# Autodesk Inventor assembly: WheelStrutLocomotion
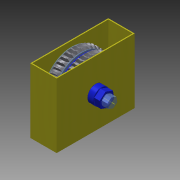
[picture p0: Inventor's stored thumbnail of the model, 180x180]
Saved by Autodesk Inventor 2014 (Build 180170000, 170)
## iProperties
Created: 2014-08-24
Part Number: WheelStrutLocomotion
Document SubType Name: Assembly
Designer: sam
Author: sam
## Documents named in this file (9)
- C:\Users\sam\Desktop\Octanis1-CAD\AI\WheelStrutLocomotion.iam
- C:\Users\sam\Desktop\Octanis1-CAD\AI\WheelStrutLocomotion\Design Accelerator\Shaft1.iam
- C:\Users\sam\Desktop\Octanis1-CAD\AI\WheelStrutLocomotion\Design Accelerator\Shaft3.iam
- C:\Users\sam\Desktop\Octanis1-CAD\AI\WheelStrutLocomotion\Design Accelerator\Worm Gears2.iam
- C:\Users\sam\Desktop\Octanis1-CAD\AI\WheelStrutLocomotion\Design Accelerator\Shaft5.iam
- C:\Users\sam\Desktop\Octanis1-CAD\AI\WheelStrutLocomotion\Design Accelerator\Worm Gears8.iam
- C:\Users\sam\Desktop\Octanis1-CAD\AI\WheelStrutLocomotion\Design Accelerator\Worm Gears9.iam
- C:\Users\sam\Desktop\Octanis1-CAD\AI\WheelStrutLocomotion\Design Accelerator\Shaft6.iam
- C:\Users\sam\Desktop\Octanis1-CAD\AI\Case.ipt
## Components (7 placed, 3 different names)
1. Shaft:1 [sub-assembly] — Cylindrical:1
2. Shaft:2 [sub-assembly] — Cylindrical:1, Mate:17
3. Shaft:4 [sub-assembly] — Mate:15, Rotational:1
4. Worm Gears:4 [sub-assembly] — Rotational:2
5. Worm Gears:5 [sub-assembly] — Rotational:1
6. Shaft:5 [sub-assembly] — Rotational:2, Mate:16
7. Case:1
## Relationships (6: Mate 3, RevoluteJoint 2, CylindricalJoint 1)
- Cylindrical:1: Shaft:1 ↔ Shaft:2
- Mate:15: Shaft:4
- Rotational:1 [RevoluteJoint] (6 mm): Shaft:4 ↔ Worm Gears:5
- Rotational:2 [RevoluteJoint] (-6 mm): Worm Gears:4 ↔ Shaft:5
- Mate:16: Shaft:5
- Mate:17: Shaft:2
